# Autodesk Inventor assembly: 조립품1
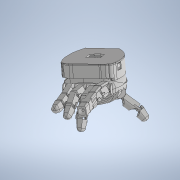
[picture p0: Inventor's stored thumbnail of the model, 180x180]
Saved by Autodesk Inventor 2022 (Build 260153000, 153)
## iProperties
Created: 2023-11-28
Part Number: 조립품1
Document SubType Name: Assembly
Designer: PC
Author: PC
## Documents named in this file (11)
- C:\Users\PC\OneDrive\바탕 화면\찐찐\조립품1.iam
- C:\Users\PC\OneDrive\바탕 화면\찐찐\뚜껑.ipt
- C:\Users\PC\OneDrive\바탕 화면\찐찐\장갑_아래_찐찐.ipt
- C:\Users\PC\OneDrive\바탕 화면\찐찐\장갑_위_찐찐.ipt
- C:\Users\PC\OneDrive\바탕 화면\찐찐\검지_손가락 위.ipt
- C:\Users\PC\OneDrive\바탕 화면\찐찐\검지_손가락아래.ipt
- C:\Users\PC\OneDrive\바탕 화면\찐찐\검지_손가락중간.ipt
- C:\Users\PC\OneDrive\바탕 화면\찐찐\손가락 위.ipt
- C:\Users\PC\OneDrive\바탕 화면\찐찐\손가락_아래.ipt
- C:\Users\PC\OneDrive\바탕 화면\찐찐\손가락_중간.ipt
- C:\Users\PC\OneDrive\바탕 화면\찐찐\센서부 90.ipt
## Components (18 placed, 10 different names)
1. 뚜껑:1 — 삽입:1, 삽입:2
2. 장갑_아래_찐찐:1 — 메이트:1, 메이트:2, 메이트:3, 메이트:7, 메이트:9, 메이트:12, 메이트:15
3. 장갑_위_찐찐:1 — 메이트:1, 메이트:2, 삽입:1, 삽입:2
4. 검지_손가락 위:1 — 메이트:5, 메이트:6
5. 검지_손가락아래:1 — 메이트:3, 메이트:4
6. 검지_손가락중간:1 — 메이트:4, 메이트:5
7. 손가락 위:1 — 메이트:11
8. 손가락_아래:1 — 메이트:7, 메이트:8
9. 손가락_중간:1 — 메이트:16, 메이트:17
10. 손가락 위:2 — 메이트:17
11. 손가락 위:3 — 메이트:14
12. 손가락 위:4 — 메이트:8
13. 손가락_아래:2 — 메이트:12, 메이트:13
14. 손가락_아래:3 — 메이트:9, 메이트:10
15. 손가락_아래:4 — 메이트:10, 메이트:11
16. 손가락_중간:2 — 메이트:13, 메이트:14
17. 손가락_중간:3 — 메이트:15, 메이트:16
18. 센서부 90:1 — 메이트:6
## Relationships (19: Mate 17, Insert 2)
- 메이트:1 [Mate]: 장갑_아래_찐찐:1 ↔ 장갑_위_찐찐:1
- 메이트:2 [Mate]: 장갑_아래_찐찐:1 ↔ 장갑_위_찐찐:1
- 삽입:1 [Insert]: 뚜껑:1 ↔ 장갑_위_찐찐:1
- 삽입:2 [Insert]: 뚜껑:1 ↔ 장갑_위_찐찐:1
- 메이트:3 [Mate]: 장갑_아래_찐찐:1 ↔ 검지_손가락아래:1
- 메이트:4 [Mate]: 검지_손가락아래:1 ↔ 검지_손가락중간:1
- 메이트:5 [Mate]: 검지_손가락 위:1 ↔ 검지_손가락중간:1
- 메이트:6 [Mate]: 검지_손가락 위:1 ↔ 센서부 90:1
- 메이트:7 [Mate]: 장갑_아래_찐찐:1 ↔ 손가락_아래:1
- 메이트:8 [Mate]: 손가락_아래:1 ↔ 손가락 위:4
- 메이트:9 [Mate]: 장갑_아래_찐찐:1 ↔ 손가락_아래:3
- 메이트:10 [Mate]: 손가락_아래:3 ↔ 손가락_아래:4
- 메이트:11 [Mate]: 손가락 위:1 ↔ 손가락_아래:4
- 메이트:12 [Mate]: 장갑_아래_찐찐:1 ↔ 손가락_아래:2
- 메이트:13 [Mate]: 손가락_아래:2 ↔ 손가락_중간:2
- 메이트:14 [Mate]: 손가락 위:3 ↔ 손가락_중간:2
- 메이트:15 [Mate]: 장갑_아래_찐찐:1 ↔ 손가락_중간:3
- 메이트:16 [Mate]: 손가락_중간:1 ↔ 손가락_중간:3
- 메이트:17 [Mate]: 손가락_중간:1 ↔ 손가락 위:2
